# Autodesk Inventor assembly: Сборка штурвал
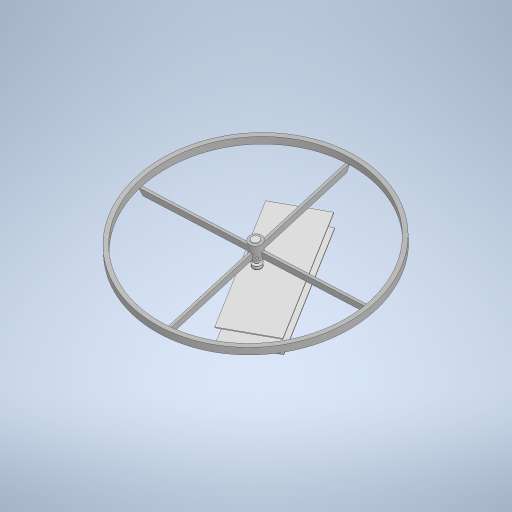
[picture p0: Inventor's stored thumbnail of the model, 512x512]
Saved by Autodesk Inventor 2023 (Build 270158000, 158)
## iProperties
Created: 2022-05-01
Part Number: Сборка штурвал
Document SubType Name: Assembly
Designer: User
Author: User
## Documents named in this file (11)
- C:\Users\avkap\Desktop\Стойка\Механизм\Сборка штурвал.iam
- C:\Users\avkap\Desktop\Стойка\Механизм\Болт маховика.ipt
- C:\Users\avkap\Desktop\Стойка\Механизм\Болт штурвал.ipt
- C:\Users\avkap\Desktop\Стойка\Механизм\Маховик.ipt
- C:\Users\avkap\Desktop\Стойка\Механизм\Вал.ipt
- C:\Users\avkap\Desktop\Стойка\Механизм\Диск (маховик, вал).ipt
- C:\Users\avkap\Desktop\Стойка\Механизм\Болт М3х16.ipt
- C:\Users\avkap\Desktop\Стойка\Механизм\Подшипник.ipt
- C:\Users\avkap\Desktop\Стойка\Механизм\Стена 16 мм отверстие.ipt
- C:\Users\avkap\Desktop\Стойка\Механизм\Штурвал.ipt
- C:\Users\avkap\Desktop\Стойка\Механизм\Part38.ipt
## Components (13 placed, 10 different names)
1. Болт маховика:1 — Совмещение:3, Совмещение:4
2. Маховик:1 — Совмещение:2, Совмещение:5, Совмещение:9, Совмещение:10, Совмещение:15
3. Вал:1 — Цилиндрический:9, Цилиндрический:10, Цилиндрический:11, Цилиндрический:12, Цилиндрический:18, Цилиндрический:19, Совмещение:12, Совмещение:13, Совмещение:16, Совмещение:17
4. Диск (маховик, вал):1 — Совмещение:6, Совмещение:7, Совмещение:8, Совмещение:10, Совмещение:11, Совмещение:13, Совмещение:15, Совмещение:16
5. Болт М3х16:3 — Совмещение:7, Совмещение:8, Совмещение:9
6. Болт М3х16:4 — Цилиндрический:9, Совмещение:6, Совмещение:11, Совмещение:12
7. Подшипник:1 — Цилиндрический:10
8. Подшипник:2 — Цилиндрический:12
9. Стена 16 мм отверстие:1 — Цилиндрический:11, Заподлицо:1
10. Стена 16 мм отверстие:2 — Цилиндрический:19, Заподлицо:1, Совмещение:18
11. Штурвал:1 — Совмещение:2, Жесткий:2, Совмещение:3, Совмещение:4, Совмещение:5
12. Part38:1 — Цилиндрический:18, Совмещение:17, Совмещение:18
13. Болт штурвал:1 — Жесткий:2
## Relationships (24: Mate 16, CylindricalJoint 6, WeldJoint 1, Flush 1)
- Цилиндрический:9 [CylindricalJoint]: Вал:1 ↔ Болт М3х16:4
- Цилиндрический:10 [CylindricalJoint]: Вал:1 ↔ Подшипник:1
- Цилиндрический:11 [CylindricalJoint]: Вал:1 ↔ Стена 16 мм отверстие:1
- Цилиндрический:12 [CylindricalJoint]: Вал:1 ↔ Подшипник:2
- Цилиндрический:18 [CylindricalJoint]: Вал:1 ↔ Part38:1
- Цилиндрический:19 [CylindricalJoint]: Вал:1 ↔ Стена 16 мм отверстие:2
- Совмещение:2 [Mate]: Маховик:1 ↔ Штурвал:1
- Жесткий:2 [WeldJoint]: Штурвал:1 ↔ Болт штурвал:1
- Совмещение:3 [Mate]: Болт маховика:1 ↔ Штурвал:1
- Совмещение:4 [Mate]: Болт маховика:1 ↔ Штурвал:1
- Совмещение:5 [Mate]: Маховик:1 ↔ Штурвал:1
- Совмещение:6 [Mate]: Диск (маховик, вал):1 ↔ Болт М3х16:4
- Совмещение:7 [Mate]: Диск (маховик, вал):1 ↔ Болт М3х16:3
- Совмещение:8 [Mate]: Диск (маховик, вал):1 ↔ Болт М3х16:3
- Совмещение:9 [Mate]: Маховик:1 ↔ Болт М3х16:3
- Совмещение:10 [Mate]: Маховик:1 ↔ Диск (маховик, вал):1
- Совмещение:11 [Mate]: Диск (маховик, вал):1 ↔ Болт М3х16:4
- Совмещение:12 [Mate]: Вал:1 ↔ Болт М3х16:4
- Совмещение:13 [Mate]: Вал:1 ↔ Диск (маховик, вал):1
- Заподлицо:1 [Flush]: Стена 16 мм отверстие:1 ↔ Стена 16 мм отверстие:2
- Совмещение:15 [Mate]: Маховик:1 ↔ Диск (маховик, вал):1
- Совмещение:16 [Mate]: Вал:1 ↔ Диск (маховик, вал):1
- Совмещение:17 [Mate]: Вал:1 ↔ Part38:1
- Совмещение:18 [Mate]: Стена 16 мм отверстие:2 ↔ Part38:1
